# Autodesk Inventor assembly: HS-100
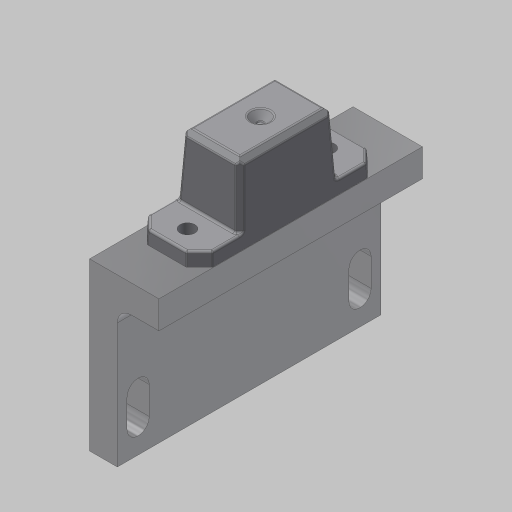
[picture p0: Inventor's stored thumbnail of the model, 512x512]
Saved by Autodesk Inventor 2023.5 (Build 275446000, 446)
## iProperties
Created: 2025-02-22
Part Number: HS-100
Document SubType Name: Assembly
Designer: slick
Author: slick
## Documents named in this file (3)
- C:\Users\slick\OneDrive\Desktop\2025-ReefScape---CAD\Elevator\Homing Sensor\HS-100.iam
- C:\Users\slick\OneDrive\Desktop\2025-ReefScape---CAD\Elevator\Homing Sensor\HS-001.ipt
- C:\Users\slick\OneDrive\Desktop\2025-ReefScape---CAD\COMMON PARTS\REV Robotics\hall effect switch assembly.iam
## Components (2 placed, 2 different names)
1. HS-001:1 — Insert:1, Insert:2
2. hall effect switch assembly:1 [sub-assembly] — Insert:1, Insert:2
## Relationships (2: Insert 2)
- Insert:1: HS-001:1 ↔ hall effect switch assembly:1
- Insert:2: HS-001:1 ↔ hall effect switch assembly:1
